# Autodesk Inventor assembly: ASY МОО 001 отстойник осветлитель
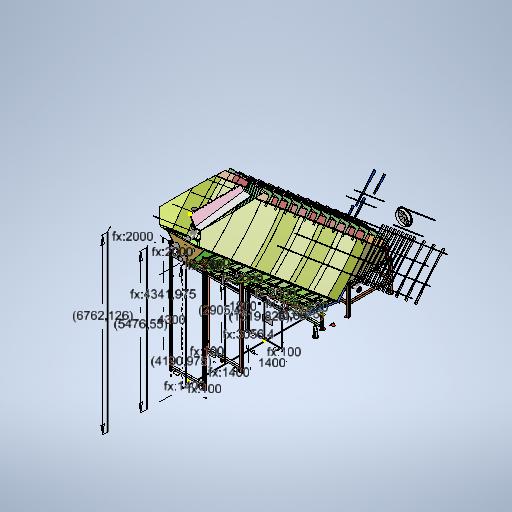
[picture p0: Inventor's stored thumbnail of the model, 512x512]
Saved by Autodesk Inventor 2025 (Build 290162010, 162A)
## iProperties
Created: 2024-04-28
Part Number: ASY МОО 001 отстойник осветлитель
Document SubType Name: Weldment
Designer: admin
Weld Material: Welded Aluminum-6061
Mass: 2.21208e+06 g
Surface Area: 2.10182e+06 cm^2
Volume: 281423 cm^3
Density: 7.86034 g/cm^3
Author: admin
## Documents named in this file (44)
- C:\Users\pokla\Documents\Inventor\Отстойник осветлитель\Manturovo_Se-clar-Gleb\ASY MSC 001 отстойник осветлитель.iam
- C:\Users\pokla\Documents\Inventor\Отстойник осветлитель\Manturovo_Se-clar-Gleb\ASY MSC 090 base frame.iam
- C:\Users\pokla\Documents\Inventor\Отстойник осветлитель\Manturovo_Se-clar-Gleb\ASY MSC 100 cone.iam
- C:\Users\pokla\Documents\Inventor\Отстойник осветлитель\Manturovo_Se-clar-Gleb\MSC 000 DIM settler-clarifier.ipt
- C:\Users\pokla\Documents\Inventor\Отстойник осветлитель\Manturovo_Se-clar-Gleb\MSC 401 sheet lowerback.ipt
- C:\Users\pokla\Documents\Inventor\Отстойник осветлитель\Manturovo_Se-clar-Gleb\MSC 313 sheet left board hip.ipt
- C:\Users\pokla\Documents\Inventor\Отстойник осветлитель\Manturovo_Se-clar-Gleb\MSC 312 sheet right board hip.ipt
- C:\Users\pokla\Documents\Inventor\Отстойник осветлитель\Manturovo_Se-clar-Gleb\MSC 706 ridge 1.ipt
- C:\Users\pokla\Documents\Inventor\Отстойник осветлитель\Manturovo_Se-clar-Gleb\MSC 705 ridge 3.ipt
- C:\Users\pokla\Documents\Inventor\Отстойник осветлитель\Manturovo_Se-clar-Gleb\MSC 701 face 1.ipt
- C:\Users\pokla\Documents\Inventor\Отстойник осветлитель\Manturovo_Se-clar-Gleb\ISO 5251 Bends 3D without straight ends(90 deg) DN150 11 11.ipt
- C:\Users\pokla\Documents\Inventor\Отстойник осветлитель\Manturovo_Se-clar-Gleb\MSC 713 tube.ipt
- C:\Users\pokla\Documents\Inventor\Отстойник осветлитель\Manturovo_Se-clar-Gleb\MSC 712 tube.ipt
- C:\Users\pokla\Documents\Inventor\Отстойник осветлитель\Manturovo_Se-clar-Gleb\MSC 711 tube.ipt
- C:\Users\pokla\Documents\Inventor\Отстойник осветлитель\Manturovo_Se-clar-Gleb\MSC 408 stringer lowerback.ipt
- C:\Users\pokla\Documents\Inventor\Отстойник осветлитель\Manturovo_Se-clar-Gleb\MSC 707 ridge 2.ipt
- C:\Users\pokla\Documents\Inventor\Отстойник осветлитель\Manturovo_Se-clar-Gleb\MSC 703 face 2.ipt
- C:\Users\pokla\Documents\Inventor\Отстойник осветлитель\Manturovo_Se-clar-Gleb\MSC 702 face 3.ipt
- C:\Users\pokla\Documents\Inventor\Отстойник осветлитель\Manturovo_Se-clar-Gleb\MSC 704 face 4.ipt
- C:\Users\pokla\Documents\Inventor\Отстойник осветлитель\Manturovo_Se-clar-Gleb\MSC 402 ring.ipt
- C:\Users\pokla\Documents\Inventor\Отстойник осветлитель\Manturovo_Se-clar-Gleb\MSC 708 ridge 4.ipt
- C:\Users\pokla\Documents\Inventor\Отстойник осветлитель\Manturovo_Se-clar-Gleb\MSC 709 ridge 5.ipt
- C:\Users\pokla\Documents\Inventor\Отстойник осветлитель\Manturovo_Se-clar-Gleb\MSC 403 flange 500.ipt
- C:\Users\pokla\Documents\Inventor\Отстойник осветлитель\Manturovo_Se-clar-Gleb\MSC 404 flange cover 500.ipt
- C:\Users\pokla\Documents\Inventor\Отстойник осветлитель\Manturovo_Se-clar-Gleb\MSC 405 flange cover ring 500.ipt
- C:\Users\pokla\Documents\Inventor\Отстойник осветлитель\Manturovo_Se-clar-Gleb\MSC 406 flange cover plate 500.ipt
- C:\Users\pokla\Documents\Inventor\Отстойник осветлитель\Manturovo_Se-clar-Gleb\ASY MSC 120  base frame.iam
- C:\Users\pokla\Documents\Inventor\Отстойник осветлитель\Manturovo_Se-clar-Gleb\Pillars\ASY MSC 900.5 base frame.iam
- C:\Users\pokla\Documents\Inventor\Отстойник осветлитель\Manturovo_Se-clar-Gleb\MSC DIM 001 frame.ipt
- C:\Users\pokla\Documents\Inventor\Отстойник осветлитель\Manturovo_Se-clar-Gleb\Pillars\ASY MSC 900.4  base frame.iam
- C:\Users\pokla\Documents\Inventor\Отстойник осветлитель\Manturovo_Se-clar-Gleb\Pillars\ASY MSC 900.6 base frame.iam
- C:\Users\pokla\Documents\Inventor\Отстойник осветлитель\Manturovo_Se-clar-Gleb\ASY MSC 201 BACK.iam
- C:\Users\pokla\Documents\Inventor\Отстойник осветлитель\Manturovo_Se-clar-Gleb\ASY MSC 202 LEFT BOARD.iam
- C:\Users\pokla\Documents\Inventor\Отстойник осветлитель\Manturovo_Se-clar-Gleb\ASY MSC 203 RIGHT BOARD.iam
- C:\Users\pokla\Documents\Inventor\Отстойник осветлитель\Manturovo_Se-clar-Gleb\ASY MSC 204 BELLY.iam
- C:\Users\pokla\Documents\Inventor\Отстойник осветлитель\Manturovo_Se-clar-Gleb\MSC 316 stringer board #.ipt
- C:\Users\pokla\Documents\Inventor\Отстойник осветлитель\Manturovo_Se-clar-Gleb\MSC 317 stringer board ##.ipt
- C:\Users\pokla\Documents\Inventor\Отстойник осветлитель\Manturovo_Se-clar-Gleb\MSC 315 rib hip.ipt
- C:\Users\pokla\Documents\Inventor\Отстойник осветлитель\Manturovo_Se-clar-Gleb\MSC 314 rib hip.ipt
- C:\Users\pokla\Documents\Inventor\Отстойник осветлитель\Manturovo_Se-clar-Gleb\ASY MSC 120 support.iam
- C:\Users\pokla\Documents\Inventor\Отстойник осветлитель\Manturovo_Se-clar-Gleb\ASY MSC 600 cone exit back.iam
- C:\Users\pokla\Documents\Inventor\Отстойник осветлитель\Manturovo_Se-clar-Gleb\MSC 710 flange.ipt
- C:\Users\pokla\Documents\Inventor\Отстойник осветлитель\Manturovo_Se-clar-Gleb\ASY MSC 800 gills.iam
- C:\Users\pokla\Documents\Inventor\Отстойник осветлитель\Manturovo_Se-clar-Gleb\MSC 407 sheet lowerback_FIX.ipt
## Components (69 placed, 43 different names)
1. MSC 000 DIM settler-clarifier.ipt:1
2. Чертеж для парам. рамы.ipt:1 — Flush:94, Mate:95
3. ASY MSC 100 cone.iam:1 [sub-assembly] — Flush:22, Mate:16, Flush:28, Mate:65, Mate:78, Flush:79, Mate:83, Flush:100
4. ASY MSC 600 cone exit back.iam:1 [sub-assembly] — Mate:140, Mate:142, Flush:101, Flush:103
5. ASY MSC 204 BELLY.iam:1 [sub-assembly] — Flush:101, Mate:144, Mate:150, Mate:151, Mate:152, Mate:153, Mate:154, Mate:158, Flush:104, Mate:159, Mate:160
6. ASY MSC 203 RIGHT BOARD.iam:1 [sub-assembly] — Mate:140, Mate:149, Mate:159, Mate:160
7. ASY MSC 202 LEFT BOARD.iam:1 [sub-assembly] — Mate:142, Flush:103
8. ASY MSC 201 BACK.iam:1 [sub-assembly] — Mate:149, Mate:158
9. ASY MSC 120 support.iam:1 [sub-assembly]
10. ASY MSC 120 support.iam:2 [sub-assembly] — Mate:152, Cylindrical:4
11. ASY MSC 120 support.iam:3 [sub-assembly]
12. ASY MSC 120 support.iam:4 [sub-assembly]
13. ASY MSC 122  base frame.iam:1 [sub-assembly]
14. ASY MSC 120.1  base frame.iam:1 [sub-assembly] — Mate:155, Mate:156, Cylindrical:3, Cylindrical:4
15. ASY MSC 121  base frame.iam:1 [sub-assembly]
16. ASY MSC 120  base frame.iam:1 [sub-assembly]
17. ASY MSC 090 base frame.iam:1 [sub-assembly] — Flush:19, Flush:21, Flush:100
18. MSC 401 sheet lowerback.ipt:1 — Mate:15, Mate:16, Tangent:10, Tangent:12
19. MSC 068 stringer lowerback.ipt:1 — Mate:65, Tangent:10
20. MSC 068 stringer lowerback.ipt:2 — Mate:83, Tangent:12
21. MSC 021 sheet left board hip.ipt:1 — Flush:41, Mate:78
22. MSC 022 sheet right board hip.ipt:1 — Mate:30
23. MSC 071 ridge 1.ipt:1 — Mate:50, Rigid:211
24. MSC 073 ridge 3.ipt:1 — Rotational:6, Rigid:210, Rigid:211
25. MSC 072 ridge 2.ipt:1 — Rotational:6
26. MSC 077 face 4.ipt:1
27. MSC 074 ridge 4.ipt:1 — Rigid:210
28. MSC 075 ridge 5.ipt:1
29. MSC 074 face 1.ipt:1 — Rigid:156, Rigid:157, Flush:62, Rigid:159, Mate:150, Mate:151
30. МОО 061 труба верх 1.ipt:1 — Rigid:59, Rigid:159
31. ISO 5251 Bends 3D without straight ends(90 deg) DN150 11 11.ipt:1 — Rigid:59, Rotational:2
32. МОО 062 труба верх 2.ipt:1 — Rigid:156
33. МОО 063 труба верх 3.ipt:1 — Rigid:157, Rigid:213
34. МОО 061 труба верх 1.ipt:2 — Rotational:2
35. MSC 075 face 2.ipt:1 — Flush:61
36. MSC 076 face 3.ipt:1 — Flush:76
37. MSC 035 ring.ipt:1 — Rigid:186
38. MSC 036 flange 500.ipt:1 — Rigid:175
39. MSC 036 flange 500.ipt:2 — Rigid:175, Rigid:176, Rigid:186
40. MSC 036 flange 500.ipt:3 — Rigid:176, Rigid:177, Mate:87
41. MSC 036 flange 500.ipt:4 — Rigid:177, Rotational:4
42. MSC 037 flange cover 500.ipt:1 — Rotational:4, Mate:87, Rigid:178, Mate:108
43. MSC 038 flange cover ring 500.ipt:1 — Rigid:178, Mate:109, Tangent:15
44. MSC 055 rib hip 2.ipt:1
45. MSC 063 stringer board #.ipt:1
46. MSC 064 stringer board ##.ipt:1
47. MSC 054 rib hip 1.ipt:1
48. MSC 063 stringer board #.ipt:2
49. MSC 054 rib hip 1.ipt:2
50. MSC 055 rib hip 2.ipt:2
51. MSC 064 stringer board ##.ipt:2
52. ASY MSC 120 support.iam:5 [sub-assembly] — Mate:153, Cylindrical:3
53. MSC 0392 flange.ipt:1 — Rigid:213
54. ASY MSC 080 gills.iam:1 [sub-assembly] — Mate:145, Mate:144
55. MSC 031 sheet lowerback_FIX.ipt:1 — Mate:146
56. ASY MSC 120 support.iam:6 [sub-assembly]
57. ASY MSC 120 support.iam:7 [sub-assembly] — Mate:154
58. MSC 039 flange cover plate 500.ipt:1 — Mate:108, Mate:109, Tangent:15
59. MSC 039 flange cover plate 500.ipt:2
60. MSC 039 flange cover plate 500.ipt:3
61. MSC 039 flange cover plate 500.ipt:4
62. MSC 039 flange cover plate 500.ipt:5
63. MSC 039 flange cover plate 500.ipt:6
64. MSC 039 flange cover plate 500.ipt:7
65. MSC 039 flange cover plate 500.ipt:8
66. MSC 039 flange cover plate 500.ipt:9
67. MSC 039 flange cover plate 500.ipt:10
68. MSC 039 flange cover plate 500.ipt:11
69. MSC 039 flange cover plate 500.ipt:12
## Component patterns: (12 elements, first: MSC 039 flange cover plate 500.ipt:1)
## Relationships (67: Mate 30, Flush 16, WeldJoint 13, Tangent 3, RevoluteJoint 3, CylindricalJoint 2)
- [Flush]: ASY MSC 201 BACK.iam:1
- Flush:19: ASY MSC 090 base frame.iam:1
- Flush:21: ASY MSC 090 base frame.iam:1
- Flush:22: ASY MSC 100 cone.iam:1
- [Flush]: ASY MSC 100 cone.iam:1
- Mate:15: MSC 401 sheet lowerback.ipt:1
- Mate:16: ASY MSC 100 cone.iam:1 ↔ MSC 401 sheet lowerback.ipt:1
- Flush:28: ASY MSC 100 cone.iam:1
- Flush:41: MSC 021 sheet left board hip.ipt:1
- Mate:30: MSC 022 sheet right board hip.ipt:1
- Mate:50 (200 mm): MSC 071 ridge 1.ipt:1
- Rigid:59 [WeldJoint]: МОО 061 труба верх 1.ipt:1 ↔ ISO 5251 Bends 3D without straight ends(90 deg) DN150 11 11.ipt:1
- Mate:65: ASY MSC 100 cone.iam:1 ↔ MSC 068 stringer lowerback.ipt:1
- [Mate]: ASY MSC 201 BACK.iam:1 ↔ MSC 068 stringer lowerback.ipt:1
- Tangent:10: MSC 401 sheet lowerback.ipt:1 ↔ MSC 068 stringer lowerback.ipt:1
- Rotational:2 [RevoluteJoint]: ISO 5251 Bends 3D without straight ends(90 deg) DN150 11 11.ipt:1 ↔ МОО 061 труба верх 1.ipt:2
- Flush:61: MSC 075 face 2.ipt:1
- Rigid:156 [WeldJoint]: MSC 074 face 1.ipt:1 ↔ МОО 062 труба верх 2.ipt:1
- Rigid:157 [WeldJoint]: MSC 074 face 1.ipt:1 ↔ МОО 063 труба верх 3.ipt:1
- Flush:62: MSC 074 face 1.ipt:1
- Rigid:159 [WeldJoint] (-200 mm): MSC 074 face 1.ipt:1 ↔ МОО 061 труба верх 1.ipt:1
- Flush:76: MSC 076 face 3.ipt:1
- Mate:78: ASY MSC 100 cone.iam:1 ↔ MSC 021 sheet left board hip.ipt:1
- Flush:79: ASY MSC 100 cone.iam:1
- Mate:83: ASY MSC 100 cone.iam:1 ↔ MSC 068 stringer lowerback.ipt:2
- [Mate]: ASY MSC 201 BACK.iam:1 ↔ MSC 068 stringer lowerback.ipt:2
- Tangent:12: MSC 401 sheet lowerback.ipt:1 ↔ MSC 068 stringer lowerback.ipt:2
- Rigid:175 [WeldJoint]: MSC 036 flange 500.ipt:1 ↔ MSC 036 flange 500.ipt:2
- Rigid:176 [WeldJoint]: MSC 036 flange 500.ipt:2 ↔ MSC 036 flange 500.ipt:3
- Rigid:177 [WeldJoint]: MSC 036 flange 500.ipt:3 ↔ MSC 036 flange 500.ipt:4
- Rotational:4 [RevoluteJoint]: MSC 036 flange 500.ipt:4 ↔ MSC 037 flange cover 500.ipt:1
- Mate:87: MSC 036 flange 500.ipt:3 ↔ MSC 037 flange cover 500.ipt:1
- Rigid:178 [WeldJoint]: MSC 037 flange cover 500.ipt:1 ↔ MSC 038 flange cover ring 500.ipt:1
- Flush:94: Чертеж для парам. рамы.ipt:1
- Mate:95: Чертеж для парам. рамы.ipt:1
- Mate:108: MSC 037 flange cover 500.ipt:1 ↔ MSC 039 flange cover plate 500.ipt:1
- Mate:109: MSC 038 flange cover ring 500.ipt:1 ↔ MSC 039 flange cover plate 500.ipt:1
- Tangent:15: MSC 038 flange cover ring 500.ipt:1 ↔ MSC 039 flange cover plate 500.ipt:1
- Rigid:186 [WeldJoint]: MSC 035 ring.ipt:1 ↔ MSC 036 flange 500.ipt:2
- [Mate]: ASY MSC 600 cone exit back.iam:1 ↔ ASY MSC 204 BELLY.iam:1
- Flush:100: ASY MSC 100 cone.iam:1 ↔ ASY MSC 090 base frame.iam:1
- [WeldJoint]: ASY MSC 100 cone.iam:1 ↔ ASY MSC 600 cone exit back.iam:1
- Rotational:6 [RevoluteJoint]: MSC 073 ridge 3.ipt:1 ↔ MSC 072 ridge 2.ipt:1
- Rigid:210 [WeldJoint]: MSC 073 ridge 3.ipt:1 ↔ MSC 074 ridge 4.ipt:1
- Rigid:211 [WeldJoint]: MSC 071 ridge 1.ipt:1 ↔ MSC 073 ridge 3.ipt:1
- Mate:140: ASY MSC 600 cone exit back.iam:1 ↔ ASY MSC 203 RIGHT BOARD.iam:1
- Mate:142: ASY MSC 600 cone exit back.iam:1 ↔ ASY MSC 202 LEFT BOARD.iam:1
- Flush:101: ASY MSC 600 cone exit back.iam:1 ↔ ASY MSC 204 BELLY.iam:1
- Flush:103: ASY MSC 600 cone exit back.iam:1 ↔ ASY MSC 202 LEFT BOARD.iam:1
- Mate:145: ASY MSC 080 gills.iam:1
- Rigid:213 [WeldJoint]: МОО 063 труба верх 3.ipt:1 ↔ MSC 0392 flange.ipt:1
- Mate:144: ASY MSC 204 BELLY.iam:1 ↔ ASY MSC 080 gills.iam:1
- Mate:146: MSC 031 sheet lowerback_FIX.ipt:1
- Mate:149: ASY MSC 203 RIGHT BOARD.iam:1 ↔ ASY MSC 201 BACK.iam:1
- Mate:150: ASY MSC 204 BELLY.iam:1 ↔ MSC 074 face 1.ipt:1
- Mate:151 (-5 mm): ASY MSC 204 BELLY.iam:1 ↔ MSC 074 face 1.ipt:1
- Mate:152: ASY MSC 204 BELLY.iam:1 ↔ ASY MSC 120 support.iam:2
- Mate:153: ASY MSC 204 BELLY.iam:1 ↔ ASY MSC 120 support.iam:5
- Mate:154: ASY MSC 204 BELLY.iam:1 ↔ ASY MSC 120 support.iam:7
- Mate:155: ASY MSC 120.1  base frame.iam:1
- Mate:156: ASY MSC 120.1  base frame.iam:1
- Cylindrical:3: ASY MSC 120.1  base frame.iam:1 ↔ ASY MSC 120 support.iam:5
- Cylindrical:4: ASY MSC 120 support.iam:2 ↔ ASY MSC 120.1  base frame.iam:1
- Mate:158 (-2860 mm): ASY MSC 204 BELLY.iam:1 ↔ ASY MSC 201 BACK.iam:1
- Flush:104: ASY MSC 204 BELLY.iam:1
- Mate:159: ASY MSC 204 BELLY.iam:1 ↔ ASY MSC 203 RIGHT BOARD.iam:1
- Mate:160 (-25 mm): ASY MSC 204 BELLY.iam:1 ↔ ASY MSC 203 RIGHT BOARD.iam:1
## Named parameters: Бак_нахлест_фланца = 25 mm, Шаг_опор_по_баку = 2000 mm
